# Autodesk Inventor assembly: FullCarV2.0
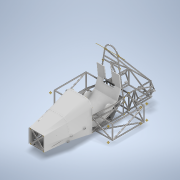
[picture p0: Inventor's stored thumbnail of the model, 180x180]
Saved by Autodesk Inventor 2021 (Build 250183000, 183)
## iProperties
Created: 2020-11-22
Part Number: FullCarV2.0
Document SubType Name: Assembly
Designer: qv17m
Author: qv17m
## Documents named in this file (15)
- C:\Users\jston\Documents\FSAE\Lafayette-Motorsports\FullCarV2.0.iam
- C:\Users\jston\Documents\FSAE\Lafayette-Motorsports\FullFrame.004\FullFrame.004.iam
- C:\Users\jston\Documents\FSAE\Lafayette-Motorsports\Drivetrain\Assembly Files\AssemblyV5.iam
- C:\Users\jston\Documents\FSAE\Lafayette-Motorsports\Seat (1).ipt
- C:\Users\jston\Documents\FSAE\Lafayette-Motorsports\SidePanels\LeftSidePanelForCar.iam
- C:\Users\jston\Documents\FSAE\Lafayette-Motorsports\SidePanels\RightSidePanelForCar.iam
- C:\Users\jston\Documents\FSAE\Lafayette-Motorsports\floorplan2\mountingtabsquareshort.ipt
- C:\Users\jston\Documents\FSAE\Lafayette-Motorsports\floorplan2\seatfloorfit.ipt
- C:\Users\jston\Documents\FSAE\Lafayette-Motorsports\floorplan2\firewalltab2.ipt
- C:\Users\jston\Documents\FSAE\Lafayette-Motorsports\floorplan2\FirewallDiagonal2.ipt
- C:\Users\jston\Documents\FSAE\Lafayette-Motorsports\floorplan2\frontfloorfit2.ipt
- C:\Users\jston\Documents\FSAE\Lafayette-Motorsports\floorplan2\angledfloorfit2.ipt
- C:\Users\jston\Documents\FSAE\Lafayette-Motorsports\FrontBody.ipt
- C:\Users\jston\Documents\FSAE\Lafayette-Motorsports\MidBody.ipt
- C:\Users\jston\Documents\FSAE\Lafayette-Motorsports\end body.ipt
## Components (26 placed, 14 different names)
1. FullFrame.004:1 [sub-assembly] — Insert:1, Angle:1, Mate:1, Mate:6, Mate:7, Mate:13, Mate:14, Mate:16, Mate:18, Mate:19, Mate:20, Mate:21, Mate:22, Mate:28, Mate:29, Mate:33, Mate:36, Mate:37, Mate:38, Mate:39, Mate:42, Tangent:1, Tangent:2, Mate:43, Mate:44, Mate:47, Mate:48, Mate:51, Mate:52, Mate:55, Mate:56, Mate:59, Mate:60
2. AssemblyV5:1 [sub-assembly] — Insert:1, Angle:1, Angle:9
3. Seat (1):1 — Angle:2
4. LeftSidePanelForCar:1 [sub-assembly]
5. RightSidePanelForCar:1 [sub-assembly]
6. mountingtabsquareshort:1 — Mate:4, Mate:5, Angle:4, Mate:6
7. mountingtabsquareshort:2 — Mate:2, Angle:3, Mate:3, Mate:7
8. mountingtabsquareshort:3 — Mate:1, Mate:8
9. seatfloorfit:1 — Mate:2, Angle:3, Mate:3, Mate:4, Mate:5, Angle:4, Mate:8, Mate:35, Angle:8
10. firewalltab2:1 — Mate:11, Mate:13
11. firewalltab2:2 — Mate:12, Mate:14, Mate:15
12. FirewallDiagonal2:1 — Mate:11, Mate:12, Mate:15, Mate:17, Mate:18
13. firewalltab2:3 — Mate:16, Mate:17
14. mountingtabsquareshort:4 — Mate:21, Mate:26
15. mountingtabsquareshort:5 — Mate:22, Mate:25
16. mountingtabsquareshort:6 — Mate:20, Mate:24, Mate:27
17. mountingtabsquareshort:7 — Mate:19, Mate:23
18. frontfloorfit2:1 — Mate:23, Mate:24, Mate:25, Mate:26, Mate:27
19. angledfloorfit2:1 — Angle:7, Mate:30, Mate:31, Mate:32, Mate:34, Mate:35
20. mountingtabsquareshort:8 — Mate:29, Mate:31, Mate:32
21. mountingtabsquareshort:9 — Mate:33, Mate:34
22. mountingtabsquareshort:10 — Angle:7
23. mountingtabsquareshort:11 — Mate:28, Mate:30
24. FrontBody:1 — Flush:3, Flush:7
25. MidBody:1 — Flush:4, Flush:5, Flush:7, Flush:8
26. end body:1 — Flush:6, Flush:8
## Relationships (78: Mate 60, Flush 8, Angle 7, Tangent 2, Insert 1)
- Insert:1 (185.547 mm): FullFrame.004:1 ↔ AssemblyV5:1
- Angle:1 (105 deg): FullFrame.004:1 ↔ AssemblyV5:1
- Angle:2 (22 deg): Seat (1):1
- Mate:1: FullFrame.004:1 ↔ mountingtabsquareshort:3
- Mate:2: mountingtabsquareshort:2 ↔ seatfloorfit:1
- Angle:3 (0 deg): mountingtabsquareshort:2 ↔ seatfloorfit:1
- Mate:3: mountingtabsquareshort:2 ↔ seatfloorfit:1
- Mate:4: mountingtabsquareshort:1 ↔ seatfloorfit:1
- Mate:5: mountingtabsquareshort:1 ↔ seatfloorfit:1
- Angle:4 (0 deg): mountingtabsquareshort:1 ↔ seatfloorfit:1
- Mate:6: FullFrame.004:1 ↔ mountingtabsquareshort:1
- Mate:7: FullFrame.004:1 ↔ mountingtabsquareshort:2
- Mate:8: mountingtabsquareshort:3 ↔ seatfloorfit:1
- Mate:11: firewalltab2:1 ↔ FirewallDiagonal2:1
- Mate:12: firewalltab2:2 ↔ FirewallDiagonal2:1
- Mate:13: FullFrame.004:1 ↔ firewalltab2:1
- Mate:14: FullFrame.004:1 ↔ firewalltab2:2
- Mate:15: firewalltab2:2 ↔ FirewallDiagonal2:1
- Mate:16: FullFrame.004:1 ↔ firewalltab2:3
- Mate:17: FirewallDiagonal2:1 ↔ firewalltab2:3
- Mate:18 (12.7 mm): FullFrame.004:1 ↔ FirewallDiagonal2:1
- Mate:19: FullFrame.004:1 ↔ mountingtabsquareshort:7
- Mate:20: FullFrame.004:1 ↔ mountingtabsquareshort:6
- Mate:21: FullFrame.004:1 ↔ mountingtabsquareshort:4
- Mate:22: FullFrame.004:1 ↔ mountingtabsquareshort:5
- Mate:23: mountingtabsquareshort:7 ↔ frontfloorfit2:1
- Mate:24: mountingtabsquareshort:6 ↔ frontfloorfit2:1
- Mate:25: mountingtabsquareshort:5 ↔ frontfloorfit2:1
- Mate:26: mountingtabsquareshort:4 ↔ frontfloorfit2:1
- Mate:27: mountingtabsquareshort:6 ↔ frontfloorfit2:1
- Angle:7 (0 deg): angledfloorfit2:1 ↔ mountingtabsquareshort:10
- Mate:28: FullFrame.004:1 ↔ mountingtabsquareshort:11
- Mate:29: FullFrame.004:1 ↔ mountingtabsquareshort:8
- Mate:30: angledfloorfit2:1 ↔ mountingtabsquareshort:11
- Mate:31: angledfloorfit2:1 ↔ mountingtabsquareshort:8
- Mate:32: angledfloorfit2:1 ↔ mountingtabsquareshort:8
- Mate:33: FullFrame.004:1 ↔ mountingtabsquareshort:9
- Mate:34: angledfloorfit2:1 ↔ mountingtabsquareshort:9
- Mate:35: seatfloorfit:1 ↔ angledfloorfit2:1
- Mate:36: FullFrame.004:1
- Mate:37: FullFrame.004:1
- Mate:38: FullFrame.004:1
- Mate:39: FullFrame.004:1
- Mate:40
- Mate:41
- Mate:42: FullFrame.004:1
- Angle:8 (0 deg): seatfloorfit:1
- Tangent:1: FullFrame.004:1
- Flush:1 (-1109.218 mm)
- Flush:2 (-132.207 mm)
- Angle:9 (0 deg): AssemblyV5:1
- Tangent:2: FullFrame.004:1
- Mate:43: FullFrame.004:1
- Mate:44: FullFrame.004:1
- Mate:45
- Mate:46
- Mate:47: FullFrame.004:1
- Mate:48: FullFrame.004:1
- Mate:49
- Mate:50
- Mate:51: FullFrame.004:1
- Mate:52: FullFrame.004:1
- Mate:53
- Mate:54
- Mate:55: FullFrame.004:1
- Mate:56: FullFrame.004:1
- Mate:57
- Mate:58
- Mate:59: FullFrame.004:1
- Mate:60: FullFrame.004:1
- Mate:61
- Mate:62
- Flush:3: FrontBody:1
- Flush:4: MidBody:1
- Flush:5: MidBody:1
- Flush:6: end body:1
- Flush:7: FrontBody:1 ↔ MidBody:1
- Flush:8: MidBody:1 ↔ end body:1
